# Autodesk Inventor assembly: Head
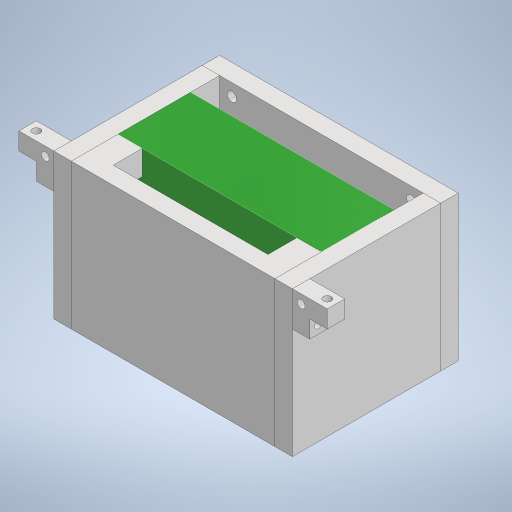
[picture p0: Inventor's stored thumbnail of the model, 512x512]
Saved by Autodesk Inventor 2024 (Build 280153000, 153)
## iProperties
Created: 2024-09-18
Part Number: Head
Document SubType Name: Assembly
Designer: Eungang
Author: Eungang
## Documents named in this file (6)
- C:\Users\Eungang\Documents\Inventor\FIGHTING_ROBOT_FINAL\부품\Head\Head.iam
- C:\Users\Eungang\Documents\Inventor\FIGHTING_ROBOT_FINAL\부품\Head\Circuit.ipt
- C:\Users\Eungang\Documents\Inventor\FIGHTING_ROBOT_FINAL\부품\Head\head_box.ipt
- C:\Users\Eungang\Documents\Inventor\FIGHTING_ROBOT_FINAL\부품\Head\head_side.ipt
- C:\Users\Eungang\Documents\Inventor\FIGHTING_ROBOT_FINAL\부품\Head\head_up.ipt
- C:\Users\Eungang\Documents\Inventor\FIGHTING_ROBOT_FINAL\부품\Head\chest_box_cap_connect.ipt
## Components (7 placed, 5 different names)
1. head_box:1 — 삽입:1, 메이트:1, 메이트:2, 메이트:3
2. Circuit:1 — 삽입:1, 플러쉬:1
3. head_side:1 — 플러쉬:1, 플러쉬:2, 메이트:4, 메이트:5, 메이트:6
4. head_side:2 — 메이트:1, 메이트:2, 메이트:3, 메이트:7, 메이트:8, 메이트:9
5. head_up:1 — 플러쉬:2
6. chest_box_cap_connect:2 — 메이트:7, 메이트:8, 메이트:9
7. chest_box_cap_connect:5 — 메이트:4, 메이트:5, 메이트:6
## Relationships (12: Mate 9, Flush 2, Insert 1)
- 삽입:1 [Insert]: head_box:1 ↔ Circuit:1
- 플러쉬:1 [Flush]: Circuit:1 ↔ head_side:1
- 메이트:1 [Mate]: head_box:1 ↔ head_side:2
- 메이트:2 [Mate]: head_box:1 ↔ head_side:2
- 메이트:3 [Mate]: head_box:1 ↔ head_side:2
- 플러쉬:2 [Flush]: head_side:1 ↔ head_up:1
- 메이트:4 [Mate]: head_side:1 ↔ chest_box_cap_connect:5
- 메이트:5 [Mate]: head_side:1 ↔ chest_box_cap_connect:5
- 메이트:6 [Mate]: head_side:1 ↔ chest_box_cap_connect:5
- 메이트:7 [Mate]: head_side:2 ↔ chest_box_cap_connect:2
- 메이트:8 [Mate]: head_side:2 ↔ chest_box_cap_connect:2
- 메이트:9 [Mate]: head_side:2 ↔ chest_box_cap_connect:2
